# Autodesk Inventor assembly: Camera pan and tilt assembly
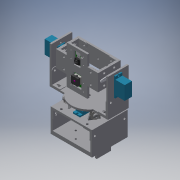
[picture p0: Inventor's stored thumbnail of the model, 180x180]
Saved by Autodesk Inventor 2018 (Build 220112000, 112)
## iProperties
Created: 2018-06-25
Part Number: Camera pan and tilt assembly
Document SubType Name: Assembly
Designer: Ajith Thomas
Author: Ajith Thomas
## Documents named in this file (16)
- C:\Users\Ajith Thomas\Dropbox\Gas_Sensing_Robot\FumeBot-Design\Pan and tilt assembly\Camera pan and tilt assembly.iam
- C:\Users\Ajith Thomas\Dropbox\Gas_Sensing_Robot\FumeBot-Design\Sensors and Boards\Raspberry Pi Camera v1.3.ipt
- C:\Users\Ajith Thomas\Dropbox\Gas_Sensing_Robot\FumeBot-Design\Pan and tilt assembly\Camera holder plate.ipt
- C:\Users\Ajith Thomas\Dropbox\Gas_Sensing_Robot\FumeBot-Design\Sensors and Boards\Lepton 3 Thermal Camera\Lepton 3 thermal camera.iam
- C:\Users\Ajith Thomas\Dropbox\Gas_Sensing_Robot\FumeBot-Design\Angle brackets\Angle bracket short.ipt
- C:\Users\Ajith Thomas\Dropbox\Gas_Sensing_Robot\FumeBot-Design\Pan and tilt assembly\Camera mount side bars.ipt
- C:\Users\Ajith Thomas\Dropbox\Gas_Sensing_Robot\FumeBot-Design\Servo motor\Servo motor.iam
- C:\Users\Ajith Thomas\Dropbox\Gas_Sensing_Robot\FumeBot-Design\Pan and tilt assembly\Camera mount raiser.ipt
- C:\Users\Ajith Thomas\Dropbox\Gas_Sensing_Robot\FumeBot-Design\Pan and tilt assembly\Camera raiser.ipt
- C:\Users\Ajith Thomas\Dropbox\Gas_Sensing_Robot\FumeBot-Design\Angle brackets\Angle bracket long.ipt
- C:\Users\Ajith Thomas\Dropbox\Gas_Sensing_Robot\FumeBot-Design\Pan and tilt assembly\Camera pan base.ipt
- C:\Users\Ajith Thomas\Dropbox\Gas_Sensing_Robot\FumeBot-Design\Pan and tilt assembly\Pan base top side bars.ipt
- C:\Users\Ajith Thomas\Dropbox\Gas_Sensing_Robot\FumeBot-Design\Pan and tilt assembly\Pan base cross bar.ipt
- C:\Users\Ajith Thomas\Dropbox\Gas_Sensing_Robot\FumeBot-Design\Pan and tilt assembly\Tilt back support with counter balance option.ipt
- C:\Users\Ajith Thomas\Dropbox\Gas_Sensing_Robot\FumeBot-Design\Pan and tilt assembly\Pan cross bar spacer.ipt
- C:\Users\Ajith Thomas\Dropbox\Gas_Sensing_Robot\FumeBot-Design\Pan and tilt assembly\Bearing Support.iam
## Components (36 placed, 15 different names)
1. Raspberry Pi Camera v1.3:1 — Flush:1, Mate:1, Flush:2
2. Camera holder plate:1 — Flush:1, Mate:2, Mate:3, Flush:3, Flush:4, Mate:4, Flush:5, Flush:6, Mate:5, Flush:7, Flush:8, Mate:6, Flush:9, Flush:10, Flush:11, Mate:7, Mate:8, Flush:12
3. Lepton 3 thermal camera:1 [sub-assembly] — Mate:1, Mate:2, Flush:2
4. Angle bracket short:1 — Mate:3, Flush:3, Flush:4
5. Angle bracket short:2 — Mate:4, Flush:5, Flush:6
6. Angle bracket short:3 — Mate:5, Flush:7, Flush:8
7. Angle bracket short:4 — Mate:6, Flush:9, Flush:10
8. Camera mount side bars:1 — Flush:11, Mate:9, Angle:1, Mate:10, Flush:26, Mate:39, Flush:27, Mate:45, Flush:30
9. Camera mount side bars:2 — Mate:7, Mate:8, Flush:12, Mate:11, Angle:2, Mate:12, Mate:41, Mate:44
10. Servo motor:1 [sub-assembly] — Mate:9, Angle:1, Mate:10, Mate:16, Mate:17, Mate:18
11. Servo motor:2 [sub-assembly] — Mate:11, Angle:2, Mate:12, Mate:13, Mate:14, Mate:15
12. Camera mount raiser:2 — Mate:13, Mate:14, Mate:15, Mate:19, Flush:14, Mate:21, Flush:15
13. Camera mount raiser:3 — Mate:16, Mate:17, Mate:18, Flush:13, Mate:23, Flush:16, Mate:25, Flush:17
14. Camera raiser:1 — Flush:13, Mate:20, Mate:22, Mate:24, Mate:26, Mate:27, Angle:3, Mate:28
15. Angle bracket long:1 — Mate:19, Flush:14, Mate:20
16. Angle bracket long:2 — Mate:21, Flush:15, Mate:22
17. Angle bracket long:3 — Mate:23, Flush:16, Mate:24
18. Angle bracket long:4 — Mate:25, Flush:17, Mate:26
19. Servo motor:3 [sub-assembly] — Mate:27, Angle:3, Mate:28, Flush:18
20. Camera pan base:1 — Flush:18, Flush:19, Mate:29, Flush:20, Mate:30, Mate:32, Flush:22, Mate:34, Mate:36, Mate:38, Mate:47, Flush:32, Flush:33
21. Pan base top side bars:1 — Flush:19, Mate:33, Flush:23, Mate:35, Flush:24
22. Pan base top side bars:2 — Mate:29, Flush:20, Mate:30, Flush:21, Mate:31, Mate:37, Flush:25
23. Pan base cross bar:1 — Flush:21, Flush:31
24. Angle bracket short:5 — Mate:31, Mate:32, Flush:22
25. Angle bracket short:6 — Mate:37, Mate:38, Flush:25
26. Angle bracket short:7 — Mate:33, Mate:34, Flush:23
27. Angle bracket short:8 — Mate:35, Mate:36, Flush:24
28. Tilt back support with counter balance option:1 — Flush:26, Mate:40, Mate:42, Flush:28, Mate:43, Flush:29, Mate:46
29. Angle bracket short:9 — Mate:39, Mate:40, Flush:27
30. Angle bracket short:10 — Mate:45, Flush:30, Mate:46
31. Angle bracket short:11 — Mate:41, Mate:42, Flush:28
32. Angle bracket short:12 — Mate:43, Flush:29, Mate:44
33. Pan cross bar spacer:1 — Flush:31
34. Bearing Support:1 [sub-assembly] — Mate:47, Flush:32, Flush:33
35. Bearing Support:2 [sub-assembly]
36. Bearing Support:3 [sub-assembly]
## Component patterns: (3 elements, first: Bearing Support:1)
## Relationships (83: Mate 47, Flush 33, Angle 3)
- Flush:1: Raspberry Pi Camera v1.3:1 ↔ Camera holder plate:1
- Mate:1 (7 mm): Raspberry Pi Camera v1.3:1 ↔ Lepton 3 thermal camera:1
- Mate:2: Camera holder plate:1 ↔ Lepton 3 thermal camera:1
- Flush:2: Raspberry Pi Camera v1.3:1 ↔ Lepton 3 thermal camera:1
- Mate:3: Camera holder plate:1 ↔ Angle bracket short:1
- Flush:3: Camera holder plate:1 ↔ Angle bracket short:1
- Flush:4: Camera holder plate:1 ↔ Angle bracket short:1
- Mate:4: Camera holder plate:1 ↔ Angle bracket short:2
- Flush:5: Camera holder plate:1 ↔ Angle bracket short:2
- Flush:6: Camera holder plate:1 ↔ Angle bracket short:2
- Mate:5: Camera holder plate:1 ↔ Angle bracket short:3
- Flush:7: Camera holder plate:1 ↔ Angle bracket short:3
- Flush:8: Camera holder plate:1 ↔ Angle bracket short:3
- Mate:6: Camera holder plate:1 ↔ Angle bracket short:4
- Flush:9: Camera holder plate:1 ↔ Angle bracket short:4
- Flush:10: Camera holder plate:1 ↔ Angle bracket short:4
- Flush:11: Camera holder plate:1 ↔ Camera mount side bars:1
- Mate:7: Camera holder plate:1 ↔ Camera mount side bars:2
- Mate:8: Camera holder plate:1 ↔ Camera mount side bars:2
- Flush:12: Camera holder plate:1 ↔ Camera mount side bars:2
- Mate:9: Camera mount side bars:1 ↔ Servo motor:1
- Angle:1 (0 deg): Camera mount side bars:1 ↔ Servo motor:1
- Mate:10: Camera mount side bars:1 ↔ Servo motor:1
- Mate:11: Camera mount side bars:2 ↔ Servo motor:2
- Angle:2 (0 deg): Camera mount side bars:2 ↔ Servo motor:2
- Mate:12: Camera mount side bars:2 ↔ Servo motor:2
- Mate:13: Servo motor:2 ↔ Camera mount raiser:2
- Mate:14: Servo motor:2 ↔ Camera mount raiser:2
- Mate:15: Servo motor:2 ↔ Camera mount raiser:2
- Mate:16: Servo motor:1 ↔ Camera mount raiser:3
- Mate:17: Servo motor:1 ↔ Camera mount raiser:3
- Mate:18: Servo motor:1 ↔ Camera mount raiser:3
- Flush:13: Camera mount raiser:3 ↔ Camera raiser:1
- Mate:19: Camera mount raiser:2 ↔ Angle bracket long:1
- Flush:14: Camera mount raiser:2 ↔ Angle bracket long:1
- Mate:20: Camera raiser:1 ↔ Angle bracket long:1
- Mate:21: Camera mount raiser:2 ↔ Angle bracket long:2
- Flush:15: Camera mount raiser:2 ↔ Angle bracket long:2
- Mate:22: Camera raiser:1 ↔ Angle bracket long:2
- Mate:23: Camera mount raiser:3 ↔ Angle bracket long:3
- Flush:16: Camera mount raiser:3 ↔ Angle bracket long:3
- Mate:24: Camera raiser:1 ↔ Angle bracket long:3
- Mate:25: Camera mount raiser:3 ↔ Angle bracket long:4
- Flush:17: Camera mount raiser:3 ↔ Angle bracket long:4
- Mate:26: Camera raiser:1 ↔ Angle bracket long:4
- Mate:27: Camera raiser:1 ↔ Servo motor:3
- Angle:3 (0 deg): Camera raiser:1 ↔ Servo motor:3
- Mate:28: Camera raiser:1 ↔ Servo motor:3
- Flush:18: Servo motor:3 ↔ Camera pan base:1
- Flush:19: Camera pan base:1 ↔ Pan base top side bars:1
- Mate:29: Camera pan base:1 ↔ Pan base top side bars:2
- Flush:20: Camera pan base:1 ↔ Pan base top side bars:2
- Mate:30: Camera pan base:1 ↔ Pan base top side bars:2
- Flush:21: Pan base top side bars:2 ↔ Pan base cross bar:1
- Mate:31: Pan base top side bars:2 ↔ Angle bracket short:5
- Mate:32: Camera pan base:1 ↔ Angle bracket short:5
- Flush:22: Camera pan base:1 ↔ Angle bracket short:5
- Mate:33: Pan base top side bars:1 ↔ Angle bracket short:7
- Mate:34: Camera pan base:1 ↔ Angle bracket short:7
- Flush:23: Pan base top side bars:1 ↔ Angle bracket short:7
- Mate:35: Pan base top side bars:1 ↔ Angle bracket short:8
- Mate:36: Camera pan base:1 ↔ Angle bracket short:8
- Flush:24: Pan base top side bars:1 ↔ Angle bracket short:8
- Mate:37: Pan base top side bars:2 ↔ Angle bracket short:6
- Mate:38: Camera pan base:1 ↔ Angle bracket short:6
- Flush:25: Pan base top side bars:2 ↔ Angle bracket short:6
- Flush:26: Camera mount side bars:1 ↔ Tilt back support with counter balance option:1
- Mate:39: Camera mount side bars:1 ↔ Angle bracket short:9
- Mate:40: Tilt back support with counter balance option:1 ↔ Angle bracket short:9
- Flush:27: Camera mount side bars:1 ↔ Angle bracket short:9
- Mate:41: Camera mount side bars:2 ↔ Angle bracket short:11
- Mate:42: Tilt back support with counter balance option:1 ↔ Angle bracket short:11
- Flush:28: Tilt back support with counter balance option:1 ↔ Angle bracket short:11
- Mate:43: Tilt back support with counter balance option:1 ↔ Angle bracket short:12
- Flush:29: Tilt back support with counter balance option:1 ↔ Angle bracket short:12
- Mate:44: Camera mount side bars:2 ↔ Angle bracket short:12
- Mate:45: Camera mount side bars:1 ↔ Angle bracket short:10
- Flush:30: Camera mount side bars:1 ↔ Angle bracket short:10
- Mate:46: Tilt back support with counter balance option:1 ↔ Angle bracket short:10
- Flush:31: Pan base cross bar:1 ↔ Pan cross bar spacer:1
- Mate:47: Camera pan base:1 ↔ Bearing Support:1
- Flush:32 (29.75 mm): Camera pan base:1 ↔ Bearing Support:1
- Flush:33 (5.7 mm): Camera pan base:1 ↔ Bearing Support:1
